# Autodesk Inventor assembly: Turntable (1544T1)
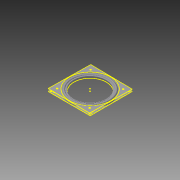
[picture p0: Inventor's stored thumbnail of the model, 180x180]
Saved by Autodesk Inventor 2015 (Build 190159000, 159)
## iProperties
Created: 2014-05-18
Part Number: Turntable (1544T1)
Document SubType Name: Assembly
Designer: seaha_000
Mass: 22.5704 g
Surface Area: 618.379 cm^2
Volume: 22.5704 cm^3
Density: 1 g/cm^3
Author: seaha_000
## Documents named in this file (7)
- X:\Dropbox\_School\AimBot\Turntable (1544T1).iam
- X:\Dropbox\_School\AimBot\Imported Components\1544T100\Part33.ipt
- X:\Dropbox\_School\AimBot\Imported Components\1544T100\Part35.ipt
- X:\Dropbox\_School\AimBot\Imported Components\1544T100\Part37.ipt
- X:\Dropbox\_School\AimBot\Imported Components\1544T100\Part39.ipt
- X:\Dropbox\_School\AimBot\Imported Components\1544T100\Part41.ipt
- X:\Dropbox\_School\AimBot\Imported Components\1544T100\Part43.ipt
## Components (6 placed, 6 different names)
1. Part33:1
2. Part35:1
3. Part37:1
4. Part39:1 — Cylindrical:1, Mate:1
5. Part41:1
6. Part43:1 — Cylindrical:1, Mate:1
## Relationships (2: CylindricalJoint 1, Mate 1)
- Cylindrical:1: Part39:1 ↔ Part43:1
- Mate:1: Part39:1 ↔ Part43:1
